# Autodesk Inventor assembly: Overall_Shooting_Mechanism2
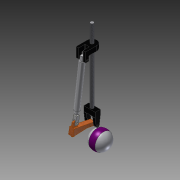
[picture p0: Inventor's stored thumbnail of the model, 180x180]
Saved by Autodesk Inventor 2015 (Build 190159000, 159)
## iProperties
Created: 2017-02-21
Part Number: Overall_Shooting_Mechanism2
Document SubType Name: Assembly
Designer: Guy
Author: Guy
## Documents named in this file (9)
- C:\Users\Guy\Documents\Fourth Year\Capstone\git\Capstone-Project\doc\CAD\SM2\Overall_Shooting_Mechanism2.iam
- C:\Users\Guy\Documents\Fourth Year\Capstone\git\Capstone-Project\doc\CAD\SM2\Swinging_connection.ipt
- C:\Users\Guy\Documents\Fourth Year\Capstone\git\Capstone-Project\doc\CAD\SM2\hinge_for_swing.ipt
- C:\Users\Guy\Documents\Fourth Year\Capstone\git\Capstone-Project\doc\CAD\ShootingMechanism\MountBar.ipt
- C:\Users\Guy\Documents\Fourth Year\Capstone\git\Capstone-Project\doc\CAD\SM2\Piston_Holder.ipt
- C:\Users\Guy\Documents\Fourth Year\Capstone\git\Capstone-Project\doc\CAD\SM2\Small_piston.ipt
- C:\Users\Guy\Documents\Fourth Year\Capstone\git\Capstone-Project\doc\CAD\SM2\piston_rod_connector.ipt
- C:\Users\Guy\Documents\Fourth Year\Capstone\git\Capstone-Project\doc\CAD\SM2\piston_internal_rod.ipt
- C:\Users\Guy\Documents\Fourth Year\Capstone\git\Capstone-Project\doc\CAD\LowLevel_Rev2\Pool_Ball_Stripe.ipt
## Components (8 placed, 8 different names)
1. hinge_for_swing:2 — Mate:3, Angle:1, Mate:7, Flush:4, Mate:14
2. MountBar:1 — Mate:3, Angle:1, Mate:6, Flush:3, Flush:4, Mate:15
3. Piston_Holder:1 — Mate:6, Mate:9, Mate:10, Flush:3
4. Swinging_connection:2 — Mate:7, Mate:11, Mate:14
5. Small_piston:1 — Mate:9, Mate:10, Mate:12, Mate:16
6. piston_rod_connector:1 — Mate:11, Flush:2, Mate:13, Mate:16
7. piston_internal_rod:1 — Mate:12, Flush:2, Mate:13
8. Pool_Ball_Stripe:1 — Mate:15
## Relationships (15: Mate 11, Flush 3, Angle 1)
- Mate:3: hinge_for_swing:2 ↔ MountBar:1
- Angle:1 (0 deg): hinge_for_swing:2 ↔ MountBar:1
- Mate:6: MountBar:1 ↔ Piston_Holder:1
- Mate:7: hinge_for_swing:2 ↔ Swinging_connection:2
- Mate:9: Piston_Holder:1 ↔ Small_piston:1
- Mate:10 (3 mm): Piston_Holder:1 ↔ Small_piston:1
- Mate:11: Swinging_connection:2 ↔ piston_rod_connector:1
- Mate:12: Small_piston:1 ↔ piston_internal_rod:1
- Flush:2: piston_rod_connector:1 ↔ piston_internal_rod:1
- Mate:13: piston_rod_connector:1 ↔ piston_internal_rod:1
- Flush:3 (-55 mm): MountBar:1 ↔ Piston_Holder:1
- Flush:4 (-5 mm): hinge_for_swing:2 ↔ MountBar:1
- Mate:14 (2.5 mm): hinge_for_swing:2 ↔ Swinging_connection:2
- Mate:15: MountBar:1 ↔ Pool_Ball_Stripe:1
- Mate:16 (3.5 mm): Small_piston:1 ↔ piston_rod_connector:1
